# Autodesk Inventor assembly: Сборка крышка
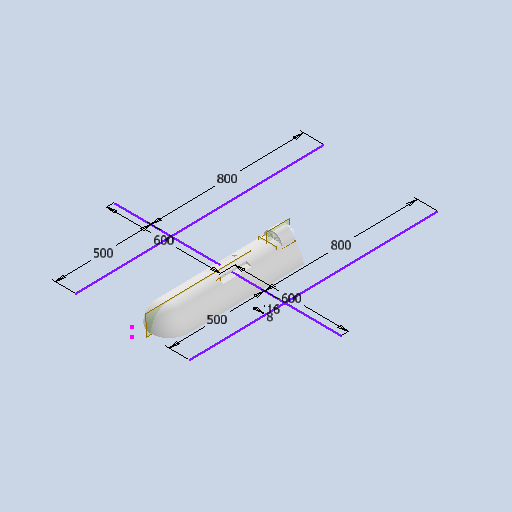
[picture p0: Inventor's stored thumbnail of the model, 512x512]
Saved by Autodesk Inventor 2022.1 (Build 261234000, 234)
## iProperties
Created: 2021-12-25
Part Number: Сборка крышка
Document SubType Name: Assembly
Designer: Grigori
Author: Grigori
## Documents named in this file (4)
- C:\Users\Grigo\Desktop\Дрон\Сборка\Сборка крышка.iam
- C:\Users\Grigo\Desktop\Дрон\Сборка\Корпус1.ipt
- C:\Users\Grigo\Desktop\Дрон\Сборка\Impeller.ipt
- C:\Users\Grigo\Desktop\Дрон\Сборка\Крышка на мотор.ipt
## Components (3 placed, 3 different names)
1. Корпус1:1 — С поворотом:1, Совмещение:1, Совмещение:2, С поворотом:3
2. Impeller:1 — С поворотом:1, С поворотом:2
3. Крышка на мотор:1 — С поворотом:2, Совмещение:1, Совмещение:2, С поворотом:3
## Relationships (5: RevoluteJoint 3, Mate 2)
- С поворотом:1 [RevoluteJoint]: Корпус1:1 ↔ Impeller:1
- С поворотом:2 [RevoluteJoint]: Impeller:1 ↔ Крышка на мотор:1
- Совмещение:1 [Mate]: Корпус1:1 ↔ Крышка на мотор:1
- Совмещение:2 [Mate]: Корпус1:1 ↔ Крышка на мотор:1
- С поворотом:3 [RevoluteJoint]: Корпус1:1 ↔ Крышка на мотор:1
